# Autodesk Inventor assembly: Сборка
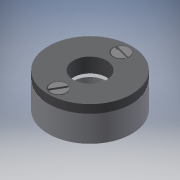
[picture p0: Inventor's stored thumbnail of the model, 180x180]
Saved by Autodesk Inventor 2019.3 (Build 233278000, 278)
## iProperties
Created: 2020-04-01
Part Number: Сборка
Material: Типовые
Document SubType Name: Assembly
Designer: Admin
Mass: 129.879 g
Surface Area: 325.125 cm^2
Volume: 129.879 cm^3
Density: 1 g/cm^3
Author: Admin
## Documents named in this file (4)
- D:\МГТУ Учеба\2 Семестр\Инжграф\Модуль 3\Сборка.iam
- D:\МГТУ Учеба\2 Семестр\Инжграф\Модуль 3\Корпус.ipt
- D:\МГТУ Учеба\2 Семестр\Инжграф\Модуль 3\Крышка.ipt
- D:\МГТУ Учеба\2 Семестр\Инжграф\Модуль 3\M8x16.ipt
## Components (4 placed, 3 different names)
1. Корпус:1 — Совмещение:1, Совмещение:2, Совмещение:3
2. Крышка:1 — Совмещение:1, Совмещение:2, Совмещение:3, Совмещение:4, Совмещение:5, Заподлицо:1, Заподлицо:2
3. M8x16:1 — Совмещение:5, Заподлицо:2
4. M8x16:2 — Совмещение:4, Заподлицо:1
## Relationships (7: Mate 5, Flush 2)
- Совмещение:1 [Mate]: Корпус:1 ↔ Крышка:1
- Совмещение:2 [Mate]: Корпус:1 ↔ Крышка:1
- Совмещение:3 [Mate]: Корпус:1 ↔ Крышка:1
- Совмещение:4 [Mate]: Крышка:1 ↔ M8x16:2
- Совмещение:5 [Mate]: Крышка:1 ↔ M8x16:1
- Заподлицо:1 [Flush]: Крышка:1 ↔ M8x16:2
- Заподлицо:2 [Flush]: Крышка:1 ↔ M8x16:1
